# Autodesk Inventor assembly: primary-engineer-bench
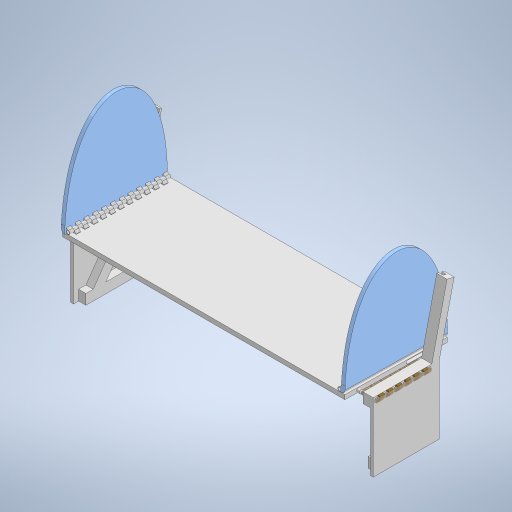
[picture p0: Inventor's stored thumbnail of the model, 512x512]
Saved by Autodesk Inventor 2023 (Build 270158030, 158C)
## iProperties
Created: 2024-09-09
Part Number: primary-engineer-bench
Document SubType Name: Assembly
Designer: Imogen Heard
Author: Imogen Heard
## Documents named in this file (7)
- C:\Users\dheard\Documents\0004-inventor\3D-CAD-main\primary-engineer-bench.iam
- C:\Users\dheard\Documents\0004-inventor\3D-CAD-main\bench-end-peice.ipt
- C:\Users\dheard\Documents\0004-inventor\3D-CAD-main\bench-slats.ipt
- C:\Users\dheard\Documents\0004-inventor\3D-CAD-main\bench-end-peice_MIR.ipt
- C:\Users\dheard\Documents\0004-inventor\3D-CAD-main\flip-up-side.ipt
- C:\Users\dheard\Documents\0004-inventor\3D-CAD-main\bed-base.ipt
- C:\Users\dheard\Documents\0004-inventor\3D-CAD-main\back-flaps-3.ipt
## Components (7 placed, 6 different names)
1. bench-end-peice:1 — Flush:1, Symmetry:1, Flush:6, lift-side-cover, Mate:1, lift-backrest
2. bench-slats:1 — Flush:1, Symmetry:1
3. bench-end-peice_MIR:1
4. flip-up-side:1 — lift-side-cover
5. bed-base:1 — Mate:1, lift-backrest, Flush:7, Mate:2, Angle:1, Rotational:3, Rotational:4
6. back-flaps-3:1 — Rotational:3
7. back-flaps-3:2 — Rotational:4
## Relationships (11: RevoluteJoint 4, Flush 3, Mate 2, Symmetry 1, Angle 1)
- Flush:1: bench-end-peice:1 ↔ bench-slats:1
- Symmetry:1: bench-end-peice:1 ↔ bench-slats:1
- Flush:6 (5 mm): bench-end-peice:1
- lift-side-cover [RevoluteJoint]: bench-end-peice:1 ↔ flip-up-side:1
- Mate:1: bench-end-peice:1 ↔ bed-base:1
- lift-backrest [RevoluteJoint]: bench-end-peice:1 ↔ bed-base:1
- Flush:7 (20 mm): bed-base:1
- Mate:2: bed-base:1
- Angle:1 (90 deg): bed-base:1
- Rotational:3 [RevoluteJoint]: bed-base:1 ↔ back-flaps-3:1
- Rotational:4 [RevoluteJoint]: bed-base:1 ↔ back-flaps-3:2
